# Autodesk Inventor assembly: Ensamblaje1
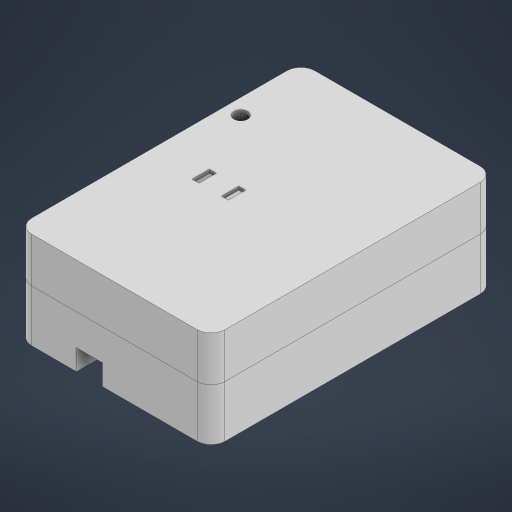
[picture p0: Inventor's stored thumbnail of the model, 512x512]
Saved by Autodesk Inventor 2023 (Build 270158000, 158)
## iProperties
Created: 2024-04-13
Part Number: Ensamblaje1
Document SubType Name: Assembly
Designer: Diego
Author: Diego
## Documents named in this file (3)
- C:\Users\Diego\Documents\CloudTechnologys\IoT\GPS\GPS_4G\Archivos 3D\Ensamblaje1.iam
- C:\Users\Diego\Documents\CloudTechnologys\IoT\GPS\GPS_4G\Archivos 3D\Pieza1.ipt
- C:\Users\Diego\Documents\CloudTechnologys\IoT\GPS\GPS_4G\Archivos 3D\Pieza2.ipt
## Components (2 placed, 2 different names)
1. Pieza1:1 — Rígido:1
2. Pieza2:1 — Rígido:1
## Relationships (1: WeldJoint 1)
- Rígido:1 [WeldJoint]: Pieza1:1 ↔ Pieza2:1
